# Autodesk Inventor assembly: IntakeMountAssembly
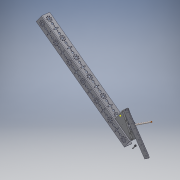
[picture p0: Inventor's stored thumbnail of the model, 180x180]
Saved by Autodesk Inventor 2017 SP1 (Build 210196100, 196)
## iProperties
Created: 2018-01-30
Part Number: IntakeMountAssembly
Document SubType Name: Assembly
Designer: 1452927
Author: 1452927
## Documents named in this file (8)
- H:\Robotics\IntakeMountAssembly.iam
- H:\Robotics\7729-CAD-master\lib\Tetrix\Structural_components\Channel 416mm.ipt
- H:\Robotics\IntakeMount.ipt
- H:\Robotics\7729-CAD-master\lib\Tetrix\Misc_Hardware\Screw SHCS 6-32 x 0.5in.ipt
- H:\Robotics\7729-CAD-master\lib\Tetrix\Axels_hubs_and_collars\Axle 100mm.ipt
- H:\Robotics\7729-CAD-master\lib\Tetrix\Axels_hubs_and_collars\Axle Set Collar.ipt
- H:\Robotics\7729-CAD-master\lib\Tetrix\Structural_components\Angle 144mm.ipt
- H:\Robotics\7729-CAD-master\lib\Tetrix\Axels_hubs_and_collars\Axle Shaft (3.7mm) Hub.ipt
## Components (7 placed, 7 different names)
1. Channel 416mm:1 — Flush:1, Mate:15, Flush:3
2. IntakeMount:1 — Flush:1, Mate:5, Mate:11, Mate:15, Flush:3, Mate:16
3. Screw SHCS 6-32 x 0.5in:1
4. Axle 100mm:1 — Mate:5, Mate:6, Flush:2, Mate:10
5. Axle Set Collar:1 — Mate:6, Flush:2, Mate:16
6. Angle 144mm:1 — Mate:12, Mate:13, Mate:14
7. Axle Shaft (3.7mm) Hub:1 — Mate:10, Mate:11, Mate:12, Mate:13, Mate:14
## Relationships (12: Mate 9, Flush 3)
- Flush:1 (2.794 mm): Channel 416mm:1 ↔ IntakeMount:1
- Mate:5: IntakeMount:1 ↔ Axle 100mm:1
- Mate:6: Axle 100mm:1 ↔ Axle Set Collar:1
- Flush:2: Axle 100mm:1 ↔ Axle Set Collar:1
- Mate:10: Axle 100mm:1 ↔ Axle Shaft (3.7mm) Hub:1
- Mate:11: IntakeMount:1 ↔ Axle Shaft (3.7mm) Hub:1
- Mate:12: Angle 144mm:1 ↔ Axle Shaft (3.7mm) Hub:1
- Mate:13: Angle 144mm:1 ↔ Axle Shaft (3.7mm) Hub:1
- Mate:14: Angle 144mm:1 ↔ Axle Shaft (3.7mm) Hub:1
- Mate:15: Channel 416mm:1 ↔ IntakeMount:1
- Flush:3: Channel 416mm:1 ↔ IntakeMount:1
- Mate:16: IntakeMount:1 ↔ Axle Set Collar:1
